# Autodesk Inventor assembly: printer
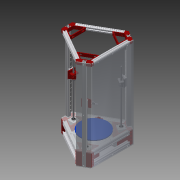
[picture p0: Inventor's stored thumbnail of the model, 180x180]
Saved by Autodesk Inventor 2015 SP1 (Build 190203100, 203)
## iProperties
Created: 2015-01-27
Part Number: printer
Document SubType Name: Assembly
Designer: Joseph
Author: Joseph
## Documents named in this file (9)
- C:\Users\Joseph\Documents\GitHub\mchp_kossel\Printer\printer.iam
- C:\Users\Joseph\Documents\GitHub\mchp_kossel\Printer\printer corner.iam
- C:\Users\Joseph\Documents\GitHub\mchp_kossel\Printer\glass.ipt
- C:\Users\Joseph\Documents\GitHub\mchp_kossel\Printer\supply.iam
- C:\Users\Joseph\Documents\GitHub\mchp_kossel\Printer\build deck.ipt
- C:\Users\Joseph\Documents\GitHub\mchp_kossel\Printer\linear stepper.iam
- C:\Users\Joseph\Documents\GitHub\mchp_kossel\Printer\small side.ipt
- C:\Users\Joseph\Documents\GitHub\mchp_kossel\Printer\large wall.ipt
- C:\Users\Joseph\Documents\GitHub\mchp_kossel\Printer\glass clamp.ipt
## Components (13 placed, 8 different names)
1. printer corner:1 [sub-assembly] — Flush:1, Flush:2, Mate:1, Mate:2, Mate:3, Mate:4, Flush:3
2. printer corner:2 [sub-assembly] — Flush:2, Mate:1, Mate:2, Mate:5, Flush:5, Flush:6
3. printer corner:3 [sub-assembly] — Flush:1, Mate:3, Mate:4, Flush:4
4. glass:1 — Mate:6
5. supply:1 [sub-assembly]
6. build deck:1 — Mate:5, Flush:3, Flush:4, Rotational:1, Cylindrical:1, Rotational:2, Rotational:3, Flush:7, Flush:8
7. linear stepper:1 [sub-assembly] — Rotational:1, Cylindrical:1
8. linear stepper:2 [sub-assembly] — Rotational:2
9. linear stepper:3 [sub-assembly] — Rotational:3
10. small side:1 — Flush:5
11. large wall:1 — Flush:6
12. glass clamp:1 — Flush:7, Flush:8, Mate:6
13. glass clamp:2
## Relationships (18: Flush 8, Mate 6, RevoluteJoint 3, CylindricalJoint 1)
- Flush:1: printer corner:1 ↔ printer corner:3
- Flush:2: printer corner:1 ↔ printer corner:2
- Mate:1: printer corner:1 ↔ printer corner:2
- Mate:2: printer corner:1 ↔ printer corner:2
- Mate:3: printer corner:1 ↔ printer corner:3
- Mate:4: printer corner:1 ↔ printer corner:3
- Mate:5: printer corner:2 ↔ build deck:1
- Flush:3: printer corner:1 ↔ build deck:1
- Flush:4: printer corner:3 ↔ build deck:1
- Rotational:1 [RevoluteJoint]: build deck:1 ↔ linear stepper:1
- Cylindrical:1: build deck:1 ↔ linear stepper:1
- Rotational:2 [RevoluteJoint]: build deck:1 ↔ linear stepper:2
- Rotational:3 [RevoluteJoint]: build deck:1 ↔ linear stepper:3
- Flush:5: printer corner:2 ↔ small side:1
- Flush:6: printer corner:2 ↔ large wall:1
- Flush:7: build deck:1 ↔ glass clamp:1
- Flush:8: build deck:1 ↔ glass clamp:1
- Mate:6: glass:1 ↔ glass clamp:1
